# Autodesk Inventor assembly: ASSY,MK4i,Swerve_Module
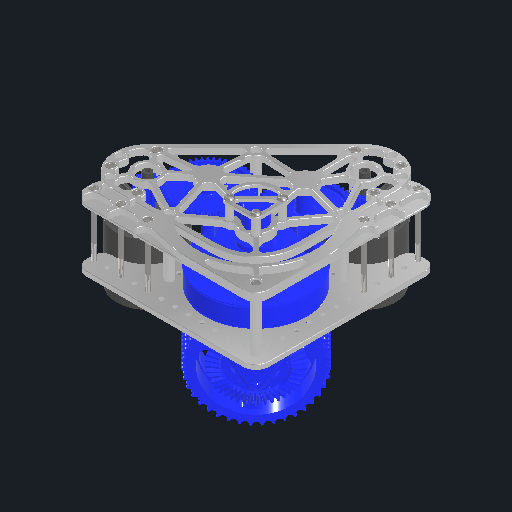
[picture p0: Inventor's stored thumbnail of the model, 512x512]
Saved by Autodesk Inventor 2023.4 (Build 274418000, 418)
## iProperties
Created: 2024-01-10
Part Number: ASSY,MK4i,Swerve_Module
Document SubType Name: Assembly
Designer: dave.simone
Author: dave.simone
## Documents named in this file (14)
- C:\Users\Johna\OneDrive - cntrline.com\FRC\FRC Library\ASSY,MK4i,Swerve_Module.iam
- C:\Users\Johna\OneDrive - cntrline.com\FRC\FRC Library\PURCHASED_SUB,PLATE,MAIN,MK4i,Swerve.ipt
- C:\Users\Johna\OneDrive - cntrline.com\FRC\FRC Library\PURCHASED_SUB,PLATE,CLAMP,MK4i,Swerve.ipt
- C:\Users\Johna\OneDrive - cntrline.com\FRC\FRC Library\PURCHASED_SUB,PLATE,UPPER,MK4i,Swerve.ipt
- C:\Users\Johna\OneDrive - cntrline.com\FRC\FRC Library\PURCHASED_SUB,PLATE,ENCODER,MK4i,Swerve.ipt
- C:\Users\Johna\OneDrive - cntrline.com\FRC\FRC Library\PURCHASED_SUB,SPACER,SHORT,MK4i,Swerve.ipt
- C:\Users\Johna\OneDrive - cntrline.com\FRC\FRC Library\PURCHASED_SUB,SPACER,LONG,MK4i,Swerve.ipt
- C:\Users\Johna\OneDrive - cntrline.com\FRC\FRC Library\SCREW,8-32 X 2.ipt
- C:\Users\Johna\OneDrive - cntrline.com\FRC\FRC Library\PURCHASED_SUB,SPACER,SHORTER,MK4i,Swerve.ipt
- C:\Users\Johna\OneDrive - cntrline.com\FRC\FRC Library\SCREW,10-32 X 1.375.ipt
- C:\Users\Johna\OneDrive - cntrline.com\FRC\FRC Library\PURCHASED_SUB,GEAR_TRAIN,WHEEL,MK4i,Swerve.ipt
- C:\Users\Johna\OneDrive - cntrline.com\FRC\FRC Library\SCREW,BUTTON,8-32 X 0.875.ipt
- C:\Users\Johna\OneDrive - cntrline.com\FRC\FRC Library\SCREW,BUTTON,10-32 X 0.250.ipt
- C:\Users\Johna\OneDrive - cntrline.com\FRC\FRC Library\CONTROLS,MOTOR,NEO,V1.ipt
## Components (41 placed, 13 different names)
1. PURCHASED_SUB,GEAR_TRAIN,WHEEL,MK4i,Swerve:1 — Mate:20, Mate:21
2. SCREW,BUTTON,8-32 X 0.875:1 — Insert:30
3. SCREW,BUTTON,8-32 X 0.875:2 — Insert:31
4. SCREW,BUTTON,8-32 X 0.875:3 — Insert:32
5. SCREW,BUTTON,10-32 X 0.250:1 — Insert:34
6. SCREW,BUTTON,10-32 X 0.250:2 — Insert:35
7. SCREW,BUTTON,10-32 X 0.250:3 — Insert:36
8. SCREW,BUTTON,10-32 X 0.250:4 — Insert:37
9. SCREW,BUTTON,10-32 X 0.250:5 — Insert:33
10. CONTROLS,MOTOR,NEO,V1:1 — Mate:22, Mate:26, Mate:27
11. CONTROLS,MOTOR,NEO,V1:2 — Mate:23, Mate:24, Mate:25
12. PURCHASED_SUB,PLATE,MAIN,MK4i,Swerve:1 — Mate:1, Mate:2, Mate:6, Mate:7, Mate:8, Mate:9, Insert:13, Mate:20, Mate:21, Insert:33, Insert:34, Insert:35, Insert:36, Insert:37, Mate:28
13. PURCHASED_SUB,PLATE,CLAMP,MK4i,Swerve:1 — Mate:1, Mate:2, Insert:14, Insert:15, Insert:16, Insert:17, Insert:18, Insert:19, Insert:23, Mate:28
14. PURCHASED_SUB,PLATE,UPPER,MK4i,Swerve:1 — Insert:4, Insert:5, Insert:6, Insert:7, Insert:8, Insert:9, Insert:10, Insert:11, Insert:12, Insert:20, Insert:21, Insert:22, Insert:24, Insert:25, Insert:26, Insert:27, Insert:28, Insert:29, Mate:22, Mate:23
15. PURCHASED_SUB,SPACER,SHORTER,MK4i,Swerve:1 — Insert:20, Mate:11
16. PURCHASED_SUB,SPACER,SHORTER,MK4i,Swerve:2 — Insert:21, Mate:12
17. PURCHASED_SUB,SPACER,SHORTER,MK4i,Swerve:3 — Insert:22, Mate:13
18. PURCHASED_SUB,SPACER,LONG,MK4i,Swerve:4 — Insert:13
19. PURCHASED_SUB,PLATE,ENCODER,MK4i,Swerve:1 — Mate:11, Mate:12, Mate:13, Insert:30, Insert:31, Insert:32
20. PURCHASED_SUB,SPACER,LONG,MK4i,Swerve:1 — Insert:4, Mate:6, Mate:7
21. PURCHASED_SUB,SPACER,LONG,MK4i,Swerve:2 — Insert:5, Mate:8
22. PURCHASED_SUB,SPACER,LONG,MK4i,Swerve:3 — Insert:6, Mate:9
23. PURCHASED_SUB,SPACER,SHORT,MK4i,Swerve:4 — Insert:8
24. PURCHASED_SUB,SPACER,SHORT,MK4i,Swerve:5 — Insert:7
25. PURCHASED_SUB,SPACER,SHORT,MK4i,Swerve:6 — Insert:9, Mate:26, Mate:27
26. PURCHASED_SUB,SPACER,SHORT,MK4i,Swerve:7 — Insert:10, Mate:24, Mate:25
27. PURCHASED_SUB,SPACER,SHORT,MK4i,Swerve:8 — Insert:11
28. PURCHASED_SUB,SPACER,SHORT,MK4i,Swerve:9 — Insert:12
29. SCREW,8-32 X 2:7 — Insert:23
30. SCREW,10-32 X 1.375:1 — Insert:24
31. SCREW,10-32 X 1.375:2 — Insert:25
32. SCREW,10-32 X 1.375:3 — Insert:26
33. SCREW,10-32 X 1.375:4 — Insert:27
34. SCREW,10-32 X 1.375:5 — Insert:28
35. SCREW,10-32 X 1.375:6 — Insert:29
36. SCREW,8-32 X 2:1 — Insert:14
37. SCREW,8-32 X 2:2 — Insert:15
38. SCREW,8-32 X 2:3 — Insert:16
39. SCREW,8-32 X 2:4 — Insert:17
40. SCREW,8-32 X 2:5 — Insert:18
41. SCREW,8-32 X 2:6 — Insert:19
## Relationships (52: Insert 34, Mate 18)
- Mate:1: PURCHASED_SUB,PLATE,MAIN,MK4i,Swerve:1 ↔ PURCHASED_SUB,PLATE,CLAMP,MK4i,Swerve:1
- Mate:2: PURCHASED_SUB,PLATE,MAIN,MK4i,Swerve:1 ↔ PURCHASED_SUB,PLATE,CLAMP,MK4i,Swerve:1
- Insert:4: PURCHASED_SUB,PLATE,UPPER,MK4i,Swerve:1 ↔ PURCHASED_SUB,SPACER,LONG,MK4i,Swerve:1
- Insert:5: PURCHASED_SUB,PLATE,UPPER,MK4i,Swerve:1 ↔ PURCHASED_SUB,SPACER,LONG,MK4i,Swerve:2
- Insert:6: PURCHASED_SUB,PLATE,UPPER,MK4i,Swerve:1 ↔ PURCHASED_SUB,SPACER,LONG,MK4i,Swerve:3
- Mate:6: PURCHASED_SUB,PLATE,MAIN,MK4i,Swerve:1 ↔ PURCHASED_SUB,SPACER,LONG,MK4i,Swerve:1
- Mate:7: PURCHASED_SUB,PLATE,MAIN,MK4i,Swerve:1 ↔ PURCHASED_SUB,SPACER,LONG,MK4i,Swerve:1
- Mate:8: PURCHASED_SUB,PLATE,MAIN,MK4i,Swerve:1 ↔ PURCHASED_SUB,SPACER,LONG,MK4i,Swerve:2
- Mate:9: PURCHASED_SUB,PLATE,MAIN,MK4i,Swerve:1 ↔ PURCHASED_SUB,SPACER,LONG,MK4i,Swerve:3
- Insert:7: PURCHASED_SUB,PLATE,UPPER,MK4i,Swerve:1 ↔ PURCHASED_SUB,SPACER,SHORT,MK4i,Swerve:5
- Insert:8: PURCHASED_SUB,PLATE,UPPER,MK4i,Swerve:1 ↔ PURCHASED_SUB,SPACER,SHORT,MK4i,Swerve:4
- Insert:9: PURCHASED_SUB,PLATE,UPPER,MK4i,Swerve:1 ↔ PURCHASED_SUB,SPACER,SHORT,MK4i,Swerve:6
- Insert:10: PURCHASED_SUB,PLATE,UPPER,MK4i,Swerve:1 ↔ PURCHASED_SUB,SPACER,SHORT,MK4i,Swerve:7
- Insert:11: PURCHASED_SUB,PLATE,UPPER,MK4i,Swerve:1 ↔ PURCHASED_SUB,SPACER,SHORT,MK4i,Swerve:8
- Insert:12: PURCHASED_SUB,PLATE,UPPER,MK4i,Swerve:1 ↔ PURCHASED_SUB,SPACER,SHORT,MK4i,Swerve:9
- Insert:13: PURCHASED_SUB,PLATE,MAIN,MK4i,Swerve:1 ↔ PURCHASED_SUB,SPACER,LONG,MK4i,Swerve:4
- Insert:14: PURCHASED_SUB,PLATE,CLAMP,MK4i,Swerve:1 ↔ SCREW,8-32 X 2:1
- Insert:15: PURCHASED_SUB,PLATE,CLAMP,MK4i,Swerve:1 ↔ SCREW,8-32 X 2:2
- Insert:16: PURCHASED_SUB,PLATE,CLAMP,MK4i,Swerve:1 ↔ SCREW,8-32 X 2:3
- Insert:17: PURCHASED_SUB,PLATE,CLAMP,MK4i,Swerve:1 ↔ SCREW,8-32 X 2:4
- Insert:18: PURCHASED_SUB,PLATE,CLAMP,MK4i,Swerve:1 ↔ SCREW,8-32 X 2:5
- Insert:19: PURCHASED_SUB,PLATE,CLAMP,MK4i,Swerve:1 ↔ SCREW,8-32 X 2:6
- Insert:20: PURCHASED_SUB,PLATE,UPPER,MK4i,Swerve:1 ↔ PURCHASED_SUB,SPACER,SHORTER,MK4i,Swerve:1
- Insert:21: PURCHASED_SUB,PLATE,UPPER,MK4i,Swerve:1 ↔ PURCHASED_SUB,SPACER,SHORTER,MK4i,Swerve:2
- Insert:22: PURCHASED_SUB,PLATE,UPPER,MK4i,Swerve:1 ↔ PURCHASED_SUB,SPACER,SHORTER,MK4i,Swerve:3
- Mate:11: PURCHASED_SUB,SPACER,SHORTER,MK4i,Swerve:1 ↔ PURCHASED_SUB,PLATE,ENCODER,MK4i,Swerve:1
- Mate:12: PURCHASED_SUB,SPACER,SHORTER,MK4i,Swerve:2 ↔ PURCHASED_SUB,PLATE,ENCODER,MK4i,Swerve:1
- Mate:13: PURCHASED_SUB,SPACER,SHORTER,MK4i,Swerve:3 ↔ PURCHASED_SUB,PLATE,ENCODER,MK4i,Swerve:1
- Insert:23: PURCHASED_SUB,PLATE,CLAMP,MK4i,Swerve:1 ↔ SCREW,8-32 X 2:7
- Insert:24: PURCHASED_SUB,PLATE,UPPER,MK4i,Swerve:1 ↔ SCREW,10-32 X 1.375:1
- Insert:25: PURCHASED_SUB,PLATE,UPPER,MK4i,Swerve:1 ↔ SCREW,10-32 X 1.375:2
- Insert:26: PURCHASED_SUB,PLATE,UPPER,MK4i,Swerve:1 ↔ SCREW,10-32 X 1.375:3
- Insert:27: PURCHASED_SUB,PLATE,UPPER,MK4i,Swerve:1 ↔ SCREW,10-32 X 1.375:4
- Insert:28: PURCHASED_SUB,PLATE,UPPER,MK4i,Swerve:1 ↔ SCREW,10-32 X 1.375:5
- Insert:29: PURCHASED_SUB,PLATE,UPPER,MK4i,Swerve:1 ↔ SCREW,10-32 X 1.375:6
- Mate:20: PURCHASED_SUB,GEAR_TRAIN,WHEEL,MK4i,Swerve:1 ↔ PURCHASED_SUB,PLATE,MAIN,MK4i,Swerve:1
- Mate:21: PURCHASED_SUB,GEAR_TRAIN,WHEEL,MK4i,Swerve:1 ↔ PURCHASED_SUB,PLATE,MAIN,MK4i,Swerve:1
- Insert:30: SCREW,BUTTON,8-32 X 0.875:1 ↔ PURCHASED_SUB,PLATE,ENCODER,MK4i,Swerve:1
- Insert:31: SCREW,BUTTON,8-32 X 0.875:2 ↔ PURCHASED_SUB,PLATE,ENCODER,MK4i,Swerve:1
- Insert:32: SCREW,BUTTON,8-32 X 0.875:3 ↔ PURCHASED_SUB,PLATE,ENCODER,MK4i,Swerve:1
- Insert:33: SCREW,BUTTON,10-32 X 0.250:5 ↔ PURCHASED_SUB,PLATE,MAIN,MK4i,Swerve:1
- Insert:34: SCREW,BUTTON,10-32 X 0.250:1 ↔ PURCHASED_SUB,PLATE,MAIN,MK4i,Swerve:1
- Insert:35: SCREW,BUTTON,10-32 X 0.250:2 ↔ PURCHASED_SUB,PLATE,MAIN,MK4i,Swerve:1
- Insert:36: SCREW,BUTTON,10-32 X 0.250:3 ↔ PURCHASED_SUB,PLATE,MAIN,MK4i,Swerve:1
- Insert:37: SCREW,BUTTON,10-32 X 0.250:4 ↔ PURCHASED_SUB,PLATE,MAIN,MK4i,Swerve:1
- Mate:22: CONTROLS,MOTOR,NEO,V1:1 ↔ PURCHASED_SUB,PLATE,UPPER,MK4i,Swerve:1
- Mate:23: CONTROLS,MOTOR,NEO,V1:2 ↔ PURCHASED_SUB,PLATE,UPPER,MK4i,Swerve:1
- Mate:24: CONTROLS,MOTOR,NEO,V1:2 ↔ PURCHASED_SUB,SPACER,SHORT,MK4i,Swerve:7
- Mate:25: CONTROLS,MOTOR,NEO,V1:2 ↔ PURCHASED_SUB,SPACER,SHORT,MK4i,Swerve:7
- Mate:26: CONTROLS,MOTOR,NEO,V1:1 ↔ PURCHASED_SUB,SPACER,SHORT,MK4i,Swerve:6
- Mate:27: CONTROLS,MOTOR,NEO,V1:1 ↔ PURCHASED_SUB,SPACER,SHORT,MK4i,Swerve:6
- Mate:28 (50.8 mm): PURCHASED_SUB,PLATE,MAIN,MK4i,Swerve:1 ↔ PURCHASED_SUB,PLATE,CLAMP,MK4i,Swerve:1
